# Autodesk Inventor assembly: door_assembly
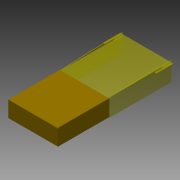
[picture p0: Inventor's stored thumbnail of the model, 180x180]
Saved by Autodesk Inventor 2014 SP2 (Build 180246200, 246)
## iProperties
Created: 2016-05-06
Part Number: door_assembly
Document SubType Name: Assembly
Designer: cruiser
Author: cruiser
## Documents named in this file (5)
- C:\Users\cruiser\Desktop\models\3d printers\laserresin4\door_assembly.iam
- C:\Users\cruiser\Desktop\models\3d printers\laserresin4\drawer.ipt
- C:\Users\cruiser\Desktop\models\3d printers\laserresin4\window.ipt
- C:\Users\cruiser\Desktop\models\3d printers\laserresin4\door.ipt
- C:\Users\cruiser\Desktop\models\3d printers\laserresin4\laserresin4.xlsx
## Components (4 placed, 3 different names)
1. drawer:1 — Mate:5, Mate:6, Mate:7, Mate:8, Flush:1, Mate:9, Flush:2
2. window:1 — Mate:7, Mate:8, Flush:1
3. window:2 — Mate:6, Mate:9, Flush:2
4. door:1 — Mate:5
## Relationships (7: Mate 5, Flush 2)
- Mate:5: drawer:1 ↔ door:1
- Mate:6: drawer:1 ↔ window:2
- Mate:7: drawer:1 ↔ window:1
- Mate:8: drawer:1 ↔ window:1
- Flush:1 (-5 mm): drawer:1 ↔ window:1
- Mate:9: drawer:1 ↔ window:2
- Flush:2 (-5 mm): drawer:1 ↔ window:2
## Named parameters: sm_thickness = 1.5875 mm, very_thick_acrylic = 9.45 mm, thick_acrylic = 5.88 mm, thin_acrylic = 3.15 mm, clear_acrylic = 3.15 mm, wood_thickness = 6.72 mm, m3_diameter = 3.15 mm, m4_diameter = 4.2 mm, m5_diameter = 5.25 mm, brass_insert_drill = 4 mm, m5_brass_insert_drill = 6.7 mm, m3_main_length = 14 mm, m3_main_nut_width = 5.7 mm, m3_main_nut_thickness = 2.5 mm, m3_main_extra = 1 mm, stepper_screw_space = 35 mm, stepper_shaft_diameter = 5 mm, stepper_body_diameter = 28 mm, laser_body_length = 40 mm, laser_body_diameter = 12 mm, carrier_x = 310 mm, carrier_y = 221 mm, carrier_z = 12 mm, visor_x = 227.3 mm, visor_y = 90.5 mm, visor_overlap = 20 mm, protection_slot = 44.2 mm, protection_slot_offset = 55.25 mm, protection_slot_length = 80 mm, window_z = 289.9125 mm, window_y = 77.0625 mm, window_overlap = 30 mm, window_slot = 50 mm, window_frame_slot = 50 mm, door_x = 221 mm, door_z = 289.9125 mm, door_overlap = 30 mm, reservoir_x = 181 mm, reservoir_y = 181 mm, reservoir_z = 50 mm, reservoir_overlap = 10 mm, linear_bearing_spacing = 247 mm, linear_bearing_z = 350 mm, threaded_rod_z = 203.2 mm, motor_spacing = 327 mm, tray_border = 20 mm, tray_x = 221 mm, tray_y = 221 mm, bed_x = 141 mm, bed_y = 141 mm, bed_z = 25.4 mm, bed_z2 = 74.6 mm, stopper_diameter = 10 mm, crane_x = 290 mm, crane_y = 70 mm, crane_z = 45 mm, crane_z2 = 12 mm, end_stop_offset_x = 47 mm, end_stop_spacing = 19 mm, acrylic_into_frame = 5 mm, protection_slot_width = 10 mm
